# Autodesk Inventor assembly: Intake_Exhaust_Assembly_2_0_2
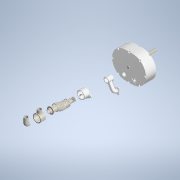
[picture p0: Inventor's stored thumbnail of the model, 180x180]
Saved by Autodesk Inventor 2021 (Build 250183000, 183)
## iProperties
Created: 2021-04-19
Part Number: Intake_Exhaust_Assembly_2_0_2
Document SubType Name: Assembly
Designer: lucia
Author: lucia
## Documents named in this file (12)
- E:\Documents\Inventor\Fixed Rotor Wankel Engine\Assemblies\Intake_Exhaust_Assembly_2_0_2.iam
- E:\Documents\Inventor\Fixed Rotor Wankel Engine\Parts\Rotor_Mount.ipt
- E:\Documents\Inventor\Fixed Rotor Wankel Engine\Parts\Eccentric_Shaft_2.ipt
- E:\Documents\Inventor\Fixed Rotor Wankel Engine\Parts\Rotor_Geared_6t_Mountable.ipt
- E:\Documents\Inventor\Fixed Rotor Wankel Engine\Parts\Side_Plate_Combined_Intake_Exhaust.ipt
- E:\Documents\Inventor\Fixed Rotor Wankel Engine\Parts\Housing.ipt
- E:\Documents\Inventor\Fixed Rotor Wankel Engine\Parts\Side_Plate_Blank.ipt
- E:\Documents\Inventor\Fixed Rotor Wankel Engine\Parts\Combined_Intake_Exhaust_Manifold.ipt
- E:\Documents\Inventor\Fixed Rotor Wankel Engine\Parts\Exhaust_Manifold_2_2.ipt
- E:\Documents\Inventor\Fixed Rotor Wankel Engine\Parts\Intake_Manifold_2.ipt
- E:\Documents\Inventor\Fixed Rotor Wankel Engine\Parts\Intake.ipt
- E:\Documents\Inventor\Fixed Rotor Wankel Engine\Parts\Exhaust.ipt
## Components (11 placed, 11 different names)
1. Rotor_Mount:1 — Mate:1, Mate:2, Mate:3, Mate:4
2. Eccentric_Shaft_2:1 — Mate:3, Mate:4, Mate:5, Mate:6, Mate:8, Mate:15, Mate:16
3. Rotor_Geared_6t_Mountable:1 — Mate:5, Mate:6, Mate:7
4. Side_Plate_Combined_Intake_Exhaust:1 — Mate:7, Mate:8, Mate:9, Mate:10, Mate:11, Mate:17, Mate:18, Mate:19, Mate:20, Mate:21, Mate:22
5. Housing:1 — Mate:9, Mate:10, Mate:11, Mate:12, Mate:13, Mate:14
6. Side_Plate_Blank:1 — Mate:12, Mate:13, Mate:14
7. Combined_Intake_Exhaust_Manifold:1 — Mate:15, Mate:16, Mate:23, Flush:1, Mate:25, Mate:26
8. Exhaust_Manifold_2_2:1 — Mate:17, Mate:18, Mate:19
9. Intake_Manifold_2:1 — Mate:20, Mate:21, Mate:22
10. Intake:1 — Mate:25, Mate:26, Mate:27
11. Exhaust:1 — Mate:23, Flush:1, Mate:24
## Relationships (28: Mate 27, Flush 1)
- Mate:1: Rotor_Mount:1
- Mate:2: Rotor_Mount:1
- Mate:3: Rotor_Mount:1 ↔ Eccentric_Shaft_2:1
- Mate:4: Rotor_Mount:1 ↔ Eccentric_Shaft_2:1
- Mate:5: Eccentric_Shaft_2:1 ↔ Rotor_Geared_6t_Mountable:1
- Mate:6: Eccentric_Shaft_2:1 ↔ Rotor_Geared_6t_Mountable:1
- Mate:7: Rotor_Geared_6t_Mountable:1 ↔ Side_Plate_Combined_Intake_Exhaust:1
- Mate:8: Eccentric_Shaft_2:1 ↔ Side_Plate_Combined_Intake_Exhaust:1
- Mate:9: Side_Plate_Combined_Intake_Exhaust:1 ↔ Housing:1
- Mate:10: Side_Plate_Combined_Intake_Exhaust:1 ↔ Housing:1
- Mate:11: Side_Plate_Combined_Intake_Exhaust:1 ↔ Housing:1
- Mate:12: Housing:1 ↔ Side_Plate_Blank:1
- Mate:13: Housing:1 ↔ Side_Plate_Blank:1
- Mate:14: Housing:1 ↔ Side_Plate_Blank:1
- Mate:15 (406.4 mm): Eccentric_Shaft_2:1 ↔ Combined_Intake_Exhaust_Manifold:1
- Mate:16: Eccentric_Shaft_2:1 ↔ Combined_Intake_Exhaust_Manifold:1
- Mate:17 (266.7 mm): Side_Plate_Combined_Intake_Exhaust:1 ↔ Exhaust_Manifold_2_2:1
- Mate:18: Side_Plate_Combined_Intake_Exhaust:1 ↔ Exhaust_Manifold_2_2:1
- Mate:19: Side_Plate_Combined_Intake_Exhaust:1 ↔ Exhaust_Manifold_2_2:1
- Mate:20 (127 mm): Side_Plate_Combined_Intake_Exhaust:1 ↔ Intake_Manifold_2:1
- Mate:21: Side_Plate_Combined_Intake_Exhaust:1 ↔ Intake_Manifold_2:1
- Mate:22: Side_Plate_Combined_Intake_Exhaust:1 ↔ Intake_Manifold_2:1
- Mate:23: Combined_Intake_Exhaust_Manifold:1 ↔ Exhaust:1
- Flush:1 (-101.6 mm): Combined_Intake_Exhaust_Manifold:1 ↔ Exhaust:1
- Mate:24: Exhaust:1
- Mate:25 (152.4 mm): Combined_Intake_Exhaust_Manifold:1 ↔ Intake:1
- Mate:26: Combined_Intake_Exhaust_Manifold:1 ↔ Intake:1
- Mate:27: Intake:1
